# Autodesk Inventor assembly: RescueKitThrow
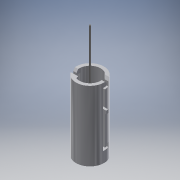
[picture p0: Inventor's stored thumbnail of the model, 180x180]
Saved by Autodesk Inventor 2018.3 (Build 223284000, 284)
## iProperties
Created: 2019-02-10
Part Number: RescueKitThrow
Material: 一般
Document SubType Name: Assembly
Designer: shun2
Author: shun2
## Documents named in this file (4)
- C:\Users\shun2\OneDrive\おそらく最新版(2018.7.31)\レスキューキット投下機構\RescueKitThrow.iam
- C:\Users\shun2\OneDrive\おそらく最新版(2018.7.31)\レスキューキット投下機構\RescueKitThrow_bottom.ipt
- C:\Users\shun2\OneDrive\おそらく最新版(2018.7.31)\レスキューキット投下機構\pianostick.ipt
- C:\Users\shun2\OneDrive\おそらく最新版(2018.7.31)\レスキューキット投下機構\RescueKitThrow_pipe.ipt
## Components (3 placed, 3 different names)
1. RescueKitThrow_bottom:1 — 円柱状:1, メイト:3
2. pianostick:1 — メイト:1, メイト:2, 円柱状:1
3. RescueKitThrow_pipe:1 — メイト:1, メイト:2, メイト:3
## Relationships (4: Mate 3, CylindricalJoint 1)
- メイト:1 [Mate]: pianostick:1 ↔ RescueKitThrow_pipe:1
- メイト:2 [Mate]: pianostick:1 ↔ RescueKitThrow_pipe:1
- 円柱状:1 [CylindricalJoint]: RescueKitThrow_bottom:1 ↔ pianostick:1
- メイト:3 [Mate]: RescueKitThrow_bottom:1 ↔ RescueKitThrow_pipe:1
